# Autodesk Inventor assembly: リンク_6_1
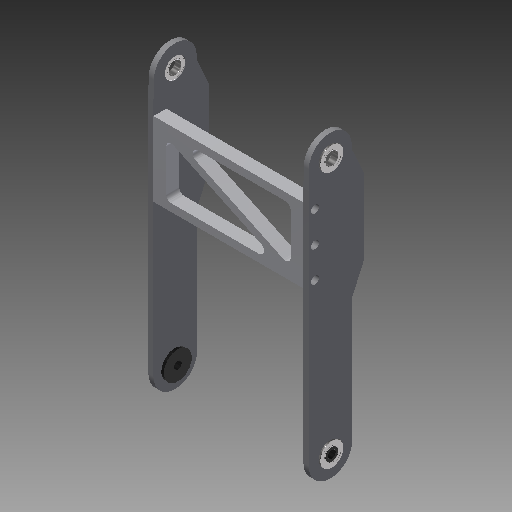
[picture p0: Inventor's stored thumbnail of the model, 512x512]
Saved by Autodesk Inventor 2018 (Build 220112000, 112)
## iProperties
Created: 2016-08-23
Part Number: リンク_6_1
Material: 一般
Document SubType Name: Assembly
Designer: hiro
Mass: 25.265 g
Surface Area: 146.992 cm^2
Volume: 11.3922 cm^3
Density: 2.21774 g/cm^3
Author: hiro
## Documents named in this file (5)
- C:\Users\taka\Documents\github\OpenPlatform\mechanism\OpenPlatform_ver3_0\下半身_160823\リンク\リンク_6_3.iam
- C:\Users\taka\Documents\github\OpenPlatform\mechanism\OpenPlatform_ver3_0\既製品\NSK_RB_MF85ZZ\MF85ZZ.iam
- C:\Users\taka\Documents\github\OpenPlatform\mechanism\OpenPlatform_ver3_0\下半身_160823\リンク\リンク_メインフレーム_6_1.ipt
- C:\Users\taka\Documents\github\OpenPlatform\mechanism\OpenPlatform_ver3_0\下半身\リンク\ふくらはぎ\リンク_ふくらはぎ_サブフレーム_1_2(予備案).ipt
- C:\Users\taka\Documents\github\OpenPlatform\mechanism\OpenPlatform_ver3_0\下半身\リンク\スペーサ\足首_スペーサ_1_1.ipt
## Components (9 placed, 4 different names)
1. MF85ZZ:1 [sub-assembly] — 挿入:34
2. MF85ZZ:2 [sub-assembly] — 挿入:29
3. MF85ZZ:3 [sub-assembly] — 挿入:33
4. MF85ZZ:4 [sub-assembly] — 挿入:28
5. リンク_メインフレーム_6_1:1 — 挿入:33, 挿入:34, 挿入:37, 挿入:38, 挿入:40
6. リンク_メインフレーム_6_1:2 — 挿入:28, 挿入:29, 挿入:35, 挿入:36, 挿入:39
7. リンク_ふくらはぎ_サブフレーム_1_2(予備案):1 — 挿入:35, 挿入:36, 挿入:37, 挿入:38
8. 足首_スペーサ_1_1:1 — 挿入:40
9. 足首_スペーサ_1_1:2 — 挿入:39
## Relationships (10: Insert 10)
- 挿入:28 [Insert]: MF85ZZ:4 ↔ リンク_メインフレーム_6_1:2
- 挿入:29 [Insert]: MF85ZZ:2 ↔ リンク_メインフレーム_6_1:2
- 挿入:33 [Insert]: MF85ZZ:3 ↔ リンク_メインフレーム_6_1:1
- 挿入:34 [Insert]: MF85ZZ:1 ↔ リンク_メインフレーム_6_1:1
- 挿入:35 [Insert]: リンク_メインフレーム_6_1:2 ↔ リンク_ふくらはぎ_サブフレーム_1_2(予備案):1
- 挿入:36 [Insert]: リンク_メインフレーム_6_1:2 ↔ リンク_ふくらはぎ_サブフレーム_1_2(予備案):1
- 挿入:37 [Insert]: リンク_メインフレーム_6_1:1 ↔ リンク_ふくらはぎ_サブフレーム_1_2(予備案):1
- 挿入:38 [Insert]: リンク_メインフレーム_6_1:1 ↔ リンク_ふくらはぎ_サブフレーム_1_2(予備案):1
- 挿入:39 [Insert]: リンク_メインフレーム_6_1:2 ↔ 足首_スペーサ_1_1:2
- 挿入:40 [Insert]: リンク_メインフレーム_6_1:1 ↔ 足首_スペーサ_1_1:1
